# Autodesk Inventor assembly: Final Assembly1
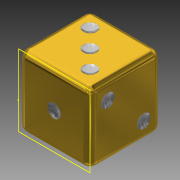
[picture p0: Inventor's stored thumbnail of the model, 180x180]
Saved by Autodesk Inventor 2013 (Build 170138000, 138)
## iProperties
Created: 2013-09-03
Part Number: Final Assembly1
Document SubType Name: Assembly
Designer: s601298
Author: s601298
## Documents named in this file (3)
- H:\School\9th Grade\IED7 Buoy, Quinn\Dice\Gold 'n silver\Final Assembly1.iam
- H:\School\9th Grade\IED7 Buoy, Quinn\Dice\Gold 'n silver\Goldnsilver die.ipt
- H:\School\9th Grade\IED7 Buoy, Quinn\Dice\Gold 'n silver\GoldPip.ipt
## Components (24 placed, 2 different names)
1. Goldnsilver die:1 — Insert:1, Insert:2, Insert:3, Insert:4, Insert:5, Insert:6, Insert:7, Insert:8, Insert:9, Insert:10, Insert:11, Insert:12, Insert:13, Insert:14, Insert:15, Insert:16, Insert:17, Insert:18, Insert:19, Insert:20, Insert:21
2. GoldPip:1
3. GoldPip:2
4. GoldPip:3 — Insert:14
5. GoldPip:4 — Insert:15
6. GoldPip:5 — Insert:18
7. GoldPip:6 — Insert:21
8. GoldPip:7 — Insert:20
9. GoldPip:8 — Insert:11
10. GoldPip:9 — Insert:6
11. GoldPip:10 — Insert:4
12. GoldPip:11 — Insert:7
13. GoldPip:12 — Insert:19
14. GoldPip:13 — Insert:17
15. GoldPip:14 — Insert:16
16. GoldPip:15 — Insert:13
17. GoldPip:16 — Insert:12
18. GoldPip:17 — Insert:10
19. GoldPip:18 — Insert:9
20. GoldPip:19 — Insert:8
21. GoldPip:20 — Insert:5
22. GoldPip:21 — Insert:3
23. GoldPip:22 — Insert:2
24. GoldPip:23 — Insert:1
## Relationships (21: Insert 21)
- Insert:1: Goldnsilver die:1 ↔ GoldPip:23
- Insert:2: Goldnsilver die:1 ↔ GoldPip:22
- Insert:3: Goldnsilver die:1 ↔ GoldPip:21
- Insert:4: Goldnsilver die:1 ↔ GoldPip:10
- Insert:5: Goldnsilver die:1 ↔ GoldPip:20
- Insert:6: Goldnsilver die:1 ↔ GoldPip:9
- Insert:7: Goldnsilver die:1 ↔ GoldPip:11
- Insert:8: Goldnsilver die:1 ↔ GoldPip:19
- Insert:9: Goldnsilver die:1 ↔ GoldPip:18
- Insert:10: Goldnsilver die:1 ↔ GoldPip:17
- Insert:11: Goldnsilver die:1 ↔ GoldPip:8
- Insert:12: Goldnsilver die:1 ↔ GoldPip:16
- Insert:13: Goldnsilver die:1 ↔ GoldPip:15
- Insert:14: Goldnsilver die:1 ↔ GoldPip:3
- Insert:15: Goldnsilver die:1 ↔ GoldPip:4
- Insert:16: Goldnsilver die:1 ↔ GoldPip:14
- Insert:17: Goldnsilver die:1 ↔ GoldPip:13
- Insert:18: Goldnsilver die:1 ↔ GoldPip:5
- Insert:19: Goldnsilver die:1 ↔ GoldPip:12
- Insert:20: Goldnsilver die:1 ↔ GoldPip:7
- Insert:21: Goldnsilver die:1 ↔ GoldPip:6
